# Autodesk Inventor assembly: mount_battery
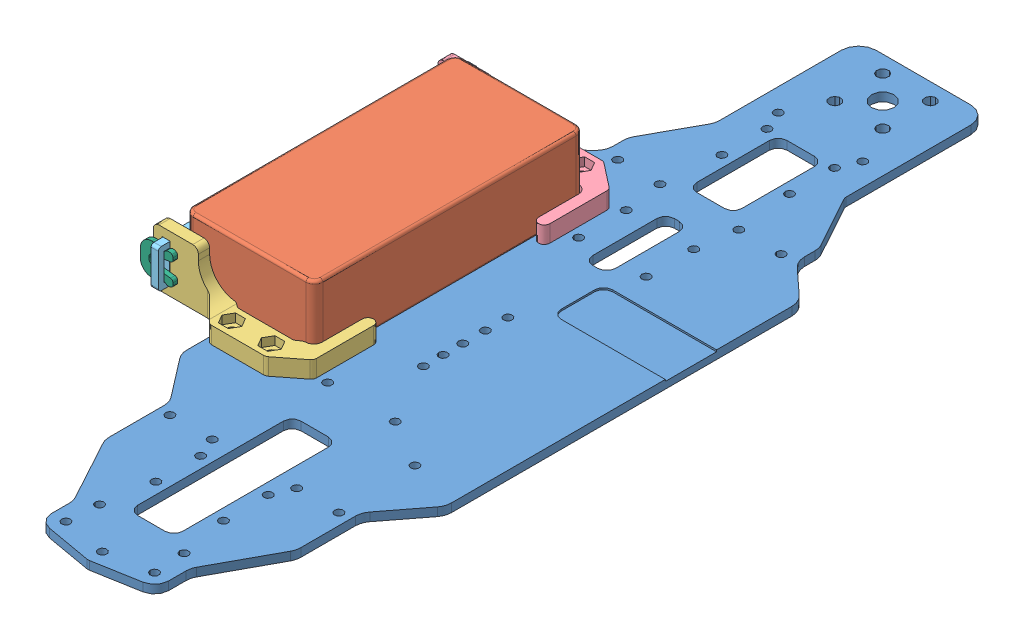
[picture p0: shaded view drawn from the shape stored in the file]
Saved by Autodesk Inventor 2021 (Build 250183000, 183)
## iProperties
Created: 2021-01-30
Part Number: mount_battery
Document SubType Name: Assembly
Designer: User
Author: User
## Documents named in this file (7)
- D:\SynologyDrive\tcodev\tco-cad\mount_battery\mount_battery.iam
- D:\SynologyDrive\tcodev\tco-cad\chassis_short\base_short.ipt
- D:\SynologyDrive\tcodev\tco-cad\common\battery.ipt
- D:\SynologyDrive\tcodev\tco-cad\mount_battery\mount_battery.ipt
- D:\SynologyDrive\tcodev\tco-cad\mount_battery\mount_battery_mirrored.ipt
- D:\SynologyDrive\tcodev\tco-cad\mount_battery\mount_battery_fastener.ipt
- D:\SynologyDrive\tcodev\tco-cad\mount_battery\fastener_clip.ipt
## Components (7 placed, 6 different names)
1. base_short:1 — Mate:1, Flush:1, Mate:2, Rigid:1
2. battery:1 — Mate:1
3. mount_battery:1 — Flush:1
4. mount_battery_mirrored:1 — Mate:2, Mate:3, Rigid:1, Mate:4, Flush:2
5. mount_battery_fastener:1 — Mate:3, Mate:4, Flush:2, Mate:10, Mate:11
6. fastener_clip:1 — Mate:10, Flush:3, Flush:4
7. fastener_clip:2 — Flush:3, Flush:4, Mate:11
## Relationships (11: Mate 6, Flush 4, WeldJoint 1)
- Mate:1: base_short:1 ↔ battery:1
- Flush:1: base_short:1 ↔ mount_battery:1
- Mate:2: base_short:1 ↔ mount_battery_mirrored:1
- Mate:3 (0.2 mm): mount_battery_mirrored:1 ↔ mount_battery_fastener:1
- Rigid:1 [WeldJoint]: base_short:1 ↔ mount_battery_mirrored:1
- Mate:4 (0.2 mm): mount_battery_mirrored:1 ↔ mount_battery_fastener:1
- Flush:2: mount_battery_mirrored:1 ↔ mount_battery_fastener:1
- Mate:10 (0.2 mm): mount_battery_fastener:1 ↔ fastener_clip:1
- Flush:3: fastener_clip:1 ↔ fastener_clip:2
- Flush:4: fastener_clip:1 ↔ fastener_clip:2
- Mate:11 (0.2 mm): mount_battery_fastener:1 ↔ fastener_clip:2
